# Autodesk Inventor assembly: Arm
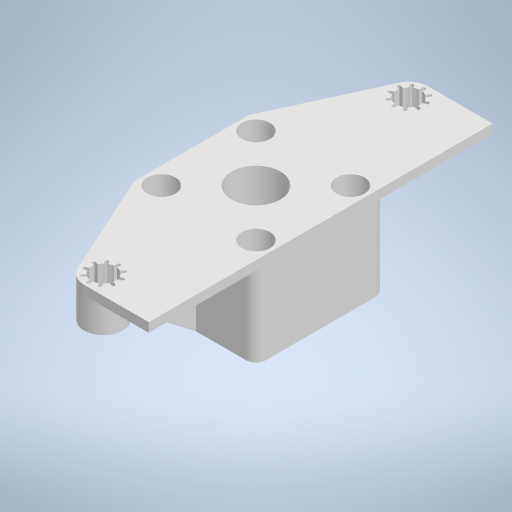
[picture p0: Inventor's stored thumbnail of the model, 512x512]
Saved by Autodesk Inventor 2024 (Build 280153000, 153)
## iProperties
Created: 2024-03-27
Part Number: Arm
Document SubType Name: Assembly
Designer: drew
Author: drew
## Documents named in this file (2)
- C:\Users\drew\Sync\CSCE 462\Arm.iam
- C:\Users\drew\Sync\CSCE 462\Arm Base stand.ipt
## Components (1 placed, 1 different names)
1. Arm Base stand:1 — Flush:1
## Relationships (1: Flush 1)
- Flush:1: Arm Base stand:1
